# Autodesk Inventor assembly: Zusammenbau
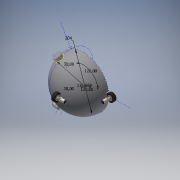
[picture p0: Inventor's stored thumbnail of the model, 180x180]
Saved by Autodesk Inventor 2017 (Build 210142000, 142)
## iProperties
Part Number: Zusammenbau
Material: Generisch
Document SubType Name: Assembly
Designer: Enno
Author: Enno
## Documents named in this file (4)
- C:\Users\Enno\Desktop\Kugelprojekt\CAD\Zusammenbau.iam
- C:\Users\Enno\Desktop\Kugelprojekt\CAD\Schale_V1.ipt
- C:\Users\Enno\Desktop\Kugelprojekt\CAD\MetallKugellager_V1.ipt
- C:\Users\Enno\Desktop\Kugelprojekt\CAD\Antrieb.iam
## Components (5 placed, 3 different names)
1. Schale_V1:1 — Passend:1, Passend:2, Fluchtend:1, Fluchtend:2, Fluchtend:3, Passend:3, Passend:4, Winkel:1, Winkel:2, Fluchtend:4, Passend:5, Passend:6, Passend:7
2. MetallKugellager_V1:1 — Passend:1, Passend:4, Winkel:2
3. MetallKugellager_V1:2 — Passend:2, Passend:3, Winkel:1
4. Antrieb:1 [sub-assembly] — Fluchtend:4, Passend:5
5. Antrieb:2 [sub-assembly] — Passend:6, Passend:7
## Relationships (13: Mate 7, Flush 4, Angle 2)
- Passend:1 [Mate]: Schale_V1:1 ↔ MetallKugellager_V1:1
- Passend:2 [Mate]: Schale_V1:1 ↔ MetallKugellager_V1:2
- Fluchtend:1 [Flush]: Schale_V1:1
- Fluchtend:2 [Flush]: Schale_V1:1
- Fluchtend:3 [Flush]: Schale_V1:1
- Passend:3 [Mate]: Schale_V1:1 ↔ MetallKugellager_V1:2
- Passend:4 [Mate]: Schale_V1:1 ↔ MetallKugellager_V1:1
- Winkel:1 [Angle] (90 deg): Schale_V1:1 ↔ MetallKugellager_V1:2
- Winkel:2 [Angle] (270 deg): Schale_V1:1 ↔ MetallKugellager_V1:1
- Fluchtend:4 [Flush]: Schale_V1:1 ↔ Antrieb:1
- Passend:5 [Mate]: Schale_V1:1 ↔ Antrieb:1
- Passend:6 [Mate]: Schale_V1:1 ↔ Antrieb:2
- Passend:7 [Mate]: Schale_V1:1 ↔ Antrieb:2
